# Autodesk Inventor assembly: assembly_linear_stepper
Saved by Autodesk Inventor 2021 (Build 250183000, 183)
## iProperties
Created: 2020-12-28
Part Number: assembly_linear_stepper
Document SubType Name: Assembly
Designer: Tomasz
Author: Tomasz
## Documents named in this file (12)
- D:\SynologyDrive\tcodev\tco-cad\camera_mount\assembly_camera_mount.iam
- D:\SynologyDrive\tcodev\tco-cad\camera_mount\linear_stepper_base.ipt
- D:\SynologyDrive\tcodev\tco-cad\camera_mount\linear_stepper_carriage.ipt
- D:\SynologyDrive\tcodev\tco-cad\camera_mount\mount_linear_stepper.ipt
- D:\SynologyDrive\tcodev\tco-cad\camera_mount\mount_carriage_top.ipt
- D:\SynologyDrive\tcodev\tco-cad\camera_mount\mount_carriage_bottom.ipt
- D:\SynologyDrive\tcodev\tco-cad\camera_mount\arm-a.ipt
- D:\SynologyDrive\tcodev\tco-cad\camera_mount\arm-b.ipt
- D:\SynologyDrive\tcodev\tco-cad\common\rod.ipt
- D:\SynologyDrive\tcodev\tco-cad\camera_mount\mount_linear_stepper_washer_b.ipt
- D:\SynologyDrive\tcodev\tco-cad\camera_mount\mount_linear_stepper_washer_a.ipt
- D:\SynologyDrive\tcodev\tco-cad\camera_mount\mount_linear_stepper_washer_c.ipt
## Components (11 placed, 11 different names)
1. linear_stepper_base:1 — Mate:1, Flush:1, Mate:2, Mate:3, Mate:4, Mate:22, Mate:23, Mate:24, Mate:25
2. linear_stepper_carriage:1 — Mate:1, Flush:1, Rigid:1, Flush:2
3. mount_linear_stepper:1 — Mate:2, Mate:3, Mate:4, Mate:14, Mate:17, Mate:19, Mate:21
4. mount_carriage_top:1 — Rigid:1, Mate:15, Mate:18
5. mount_carriage_bottom:1 — Flush:2
6. rod:1 — Mate:14
7. arm-a:1 — Mate:15, Mate:18, Mate:20
8. arm-b:1 — Mate:17, Mate:19, Mate:20
9. mount_linear_stepper_washer_b:1 — Mate:24
10. mount_linear_stepper_washer_a:1 — Mate:21, Mate:22, Mate:23
11. mount_linear_stepper_washer_c:1 — Mate:25
## Relationships (18: Mate 15, Flush 2, WeldJoint 1)
- Mate:1: linear_stepper_base:1 ↔ linear_stepper_carriage:1
- Flush:1: linear_stepper_base:1 ↔ linear_stepper_carriage:1
- Mate:2: linear_stepper_base:1 ↔ mount_linear_stepper:1
- Mate:3: linear_stepper_base:1 ↔ mount_linear_stepper:1
- Mate:4: linear_stepper_base:1 ↔ mount_linear_stepper:1
- Rigid:1 [WeldJoint]: linear_stepper_carriage:1 ↔ mount_carriage_top:1
- Flush:2: linear_stepper_carriage:1 ↔ mount_carriage_bottom:1
- Mate:14: mount_linear_stepper:1 ↔ rod:1
- Mate:15: mount_carriage_top:1 ↔ arm-a:1
- Mate:17: mount_linear_stepper:1 ↔ arm-b:1
- Mate:18: mount_carriage_top:1 ↔ arm-a:1
- Mate:19: mount_linear_stepper:1 ↔ arm-b:1
- Mate:20: arm-a:1 ↔ arm-b:1
- Mate:21: mount_linear_stepper:1 ↔ mount_linear_stepper_washer_a:1
- Mate:22: linear_stepper_base:1 ↔ mount_linear_stepper_washer_a:1
- Mate:23: linear_stepper_base:1 ↔ mount_linear_stepper_washer_a:1
- Mate:24: linear_stepper_base:1 ↔ mount_linear_stepper_washer_b:1
- Mate:25: linear_stepper_base:1 ↔ mount_linear_stepper_washer_c:1
